# Autodesk Inventor assembly: FullShortRobot
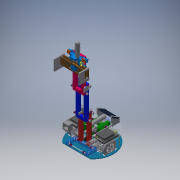
[picture p0: Inventor's stored thumbnail of the model, 180x180]
Saved by Autodesk Inventor 2019 (Build 230136000, 136)
## iProperties
Created: 2019-09-28
Part Number: FullShortRobot
Document SubType Name: Assembly
Designer: james
Author: james
## Documents named in this file (7)
- F:\JimsDesign\Jims2020FTC\FullShortRobot.iam
- F:\JimsDesign\Jims2020FTC\FullBottom.iam
- F:\JimsDesign\Library\McMaster\SocketScrews\91251A197_BLACK-OXIDE ALLOY STEEL SOCKET HEAD CAP SCREW.ipt
- F:\JimsDesign\Jims2020FTC\TopOfRobot.iam
- F:\JimsDesign\Library\McMaster\SocketScrews\91251A201_BLACK-OXIDE ALLOY STEEL SOCKET HEAD SCREW.ipt
- F:\JimsDesign\Jims2020FTC\CameraMount v4.ipt
- F:\JimsDesign\Jims2020FTC\FullShortElevator.iam
## Components (10 placed, 6 different names)
1. FullBottom:1 [sub-assembly] — Mate:2, Mate:5, Mate:6, Mate:8, Mate:13, Mate:17, Mate:18, Mate:19, Mate:20, Mate:21, Mate:22, Mate:23, Mate:24, Mate:25, Mate:28
2. FullShortElevator:1 [sub-assembly] — Mate:15, Mate:16, Mate:17
3. 91251A197_BLACK-OXIDE ALLOY STEEL SOCKET HEAD CAP SCREW:1 — Mate:5, Mate:8, Mate:16
4. 91251A197_BLACK-OXIDE ALLOY STEEL SOCKET HEAD CAP SCREW:4 — Mate:2, Mate:6, Mate:15
5. TopOfRobot:1 [sub-assembly] — Mate:13, Mate:26, Flush:1, Mate:28
6. 91251A201_BLACK-OXIDE ALLOY STEEL SOCKET HEAD SCREW:1 — Mate:21, Mate:24
7. 91251A201_BLACK-OXIDE ALLOY STEEL SOCKET HEAD SCREW:2 — Mate:20, Mate:25
8. 91251A201_BLACK-OXIDE ALLOY STEEL SOCKET HEAD SCREW:3 — Mate:19, Mate:23
9. 91251A201_BLACK-OXIDE ALLOY STEEL SOCKET HEAD SCREW:4 — Mate:18, Mate:22
10. CameraMount v4:1 — Mate:26, Flush:1
## Relationships (19: Mate 18, Flush 1)
- Mate:2: FullBottom:1 ↔ 91251A197_BLACK-OXIDE ALLOY STEEL SOCKET HEAD CAP SCREW:4
- Mate:5: FullBottom:1 ↔ 91251A197_BLACK-OXIDE ALLOY STEEL SOCKET HEAD CAP SCREW:1
- Mate:6: FullBottom:1 ↔ 91251A197_BLACK-OXIDE ALLOY STEEL SOCKET HEAD CAP SCREW:4
- Mate:8: FullBottom:1 ↔ 91251A197_BLACK-OXIDE ALLOY STEEL SOCKET HEAD CAP SCREW:1
- Mate:13: FullBottom:1 ↔ TopOfRobot:1
- Mate:15: FullShortElevator:1 ↔ 91251A197_BLACK-OXIDE ALLOY STEEL SOCKET HEAD CAP SCREW:4
- Mate:16: FullShortElevator:1 ↔ 91251A197_BLACK-OXIDE ALLOY STEEL SOCKET HEAD CAP SCREW:1
- Mate:17: FullBottom:1 ↔ FullShortElevator:1
- Mate:18: FullBottom:1 ↔ 91251A201_BLACK-OXIDE ALLOY STEEL SOCKET HEAD SCREW:4
- Mate:19: FullBottom:1 ↔ 91251A201_BLACK-OXIDE ALLOY STEEL SOCKET HEAD SCREW:3
- Mate:20: FullBottom:1 ↔ 91251A201_BLACK-OXIDE ALLOY STEEL SOCKET HEAD SCREW:2
- Mate:21: FullBottom:1 ↔ 91251A201_BLACK-OXIDE ALLOY STEEL SOCKET HEAD SCREW:1
- Mate:22: FullBottom:1 ↔ 91251A201_BLACK-OXIDE ALLOY STEEL SOCKET HEAD SCREW:4
- Mate:23: FullBottom:1 ↔ 91251A201_BLACK-OXIDE ALLOY STEEL SOCKET HEAD SCREW:3
- Mate:24: FullBottom:1 ↔ 91251A201_BLACK-OXIDE ALLOY STEEL SOCKET HEAD SCREW:1
- Mate:25: FullBottom:1 ↔ 91251A201_BLACK-OXIDE ALLOY STEEL SOCKET HEAD SCREW:2
- Mate:26: TopOfRobot:1 ↔ CameraMount v4:1
- Flush:1: TopOfRobot:1 ↔ CameraMount v4:1
- Mate:28: FullBottom:1 ↔ TopOfRobot:1
